# Autodesk Inventor assembly: VertV2
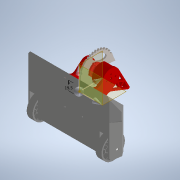
[picture p0: Inventor's stored thumbnail of the model, 180x180]
Saved by Autodesk Inventor 2020 (Build 240168000, 168)
## iProperties
Created: 2024-02-19
Part Number: VertV2
Document SubType Name: Assembly
Designer: smz3rm
Mass: 425.79 g
Surface Area: 1620.3 cm^2
Volume: 318.186 cm^3
Density: 1.33818 g/cm^3
Author: smz3rm
## Documents named in this file (7)
- C:\Users\smz3rm\OneDrive - BP\Documents\Battlebots\VerticalSpinner\VertV2.iam
- C:\Users\smz3rm\OneDrive - BP\Documents\Battlebots\VerticalSpinner\WeaponAndMount.iam
- C:\Users\smz3rm\OneDrive - BP\Documents\Battlebots\VerticalSpinner\VertBodyV2.ipt
- C:\Users\smz3rm\OneDrive - BP\Documents\Battlebots\VerticalSpinner\DriveSystem.iam
- C:\Users\smz3rm\OneDrive - BP\Documents\Battlebots\BatteryV1.ipt
- C:\Users\smz3rm\OneDrive - BP\Documents\Battlebots\FS2A.ipt
- C:\Users\smz3rm\OneDrive - BP\Documents\Battlebots\Switch.ipt
## Components (7 placed, 6 different names)
1. WeaponAndMount:1 [sub-assembly] — Mate:1, Mate:2, Mate:3, Mate:13
2. VertBodyV2:1 — Mate:1, Mate:2, Mate:3, Mate:4, Mate:5, Mate:6, Mate:7, Mate:8, Mate:9, Mate:10, Mate:11, Mate:12, Mate:14, Mate:15
3. DriveSystem:1 [sub-assembly] — Mate:6, Mate:7
4. DriveSystem:2 [sub-assembly] — Mate:4, Mate:5
5. BatteryV1:1 — Mate:8, Mate:9, Mate:10
6. FS2A:1 — Mate:11
7. Switch:1 — Mate:12
## Relationships (15: Mate 15)
- Mate:1: WeaponAndMount:1 ↔ VertBodyV2:1
- Mate:2: WeaponAndMount:1 ↔ VertBodyV2:1
- Mate:3: WeaponAndMount:1 ↔ VertBodyV2:1
- Mate:4: VertBodyV2:1 ↔ DriveSystem:2
- Mate:5: VertBodyV2:1 ↔ DriveSystem:2
- Mate:6: VertBodyV2:1 ↔ DriveSystem:1
- Mate:7: VertBodyV2:1 ↔ DriveSystem:1
- Mate:8: VertBodyV2:1 ↔ BatteryV1:1
- Mate:9: VertBodyV2:1 ↔ BatteryV1:1
- Mate:10: VertBodyV2:1 ↔ BatteryV1:1
- Mate:11: VertBodyV2:1 ↔ FS2A:1
- Mate:12: VertBodyV2:1 ↔ Switch:1
- Mate:13: WeaponAndMount:1
- Mate:14: VertBodyV2:1
- Mate:15: VertBodyV2:1
